# Autodesk Inventor assembly: Deltabot - Small Model ver12
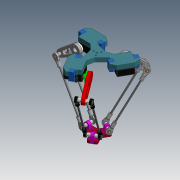
[picture p0: Inventor's stored thumbnail of the model, 180x180]
Saved by Autodesk Inventor 2014 SP1 (Build 180222100, 222)
## iProperties
Created: 2013-12-25
Part Number: Deltabot - Small Model ver12
Document SubType Name: Assembly
Designer: tom
Title: D:\My Documents\Work\GitHub\Delta_Robots\Delatabot - Small Model\Deltabot - Small Model.stp
Creation Date: 2013-12-24
Sending System: ACIS
Author: tom
## Documents named in this file (7)
- C:\Users\tom\Documents\GitHub\Delta_Robots\Delatabot - Small Model\Inventor\Deltabot - Small Model ver12\Deltabot - Small Model ver12.iam
- C:\Users\tom\Documents\GitHub\Vacubot\Inventor\Part2.ipt
- C:\Users\tom\Documents\GitHub\Delta_Robots\Delatabot - Small Model\Inventor\Deltabot - Small Model ver12\Servo_Mount.ipt
- C:\Users\tom\Documents\GitHub\Delta_Robots\Delatabot - Small Model\Inventor\Deltabot - Small Model ver12\Servo.ipt
- C:\Users\tom\Documents\GitHub\Delta_Robots\Delatabot - Small Model\Inventor\Deltabot - Small Model ver12\Servo Arm.iam
- C:\Users\tom\Documents\GitHub\Delta_Robots\Delatabot - Small Model\Inventor\Deltabot - Small Model ver12\Arm Linkage.iam
- C:\Users\tom\Documents\GitHub\Delta_Robots\Delatabot - Small Model\Inventor\Deltabot - Small Model ver12\Lower Platform Assembly.iam
## Components (20 placed, 6 different names)
1. Upper Support — Mate:15, Mate:16, Mate:17, Mate:19
2. Servo Arm:1 [sub-assembly] — Ball:1, Ball:3
3. Arm Linkage:1 [sub-assembly] — Ball:1, Ball:2
4. Lower Platform Assembly:1 [sub-assembly] — Ball:2, Ball:4, Ball:6, Ball:8, Ball:10, Ball:12
5. Arm Linkage:2 [sub-assembly] — Ball:3, Ball:4
6. Servo Arm:2 [sub-assembly] — Rotational:2, Ball:5, Ball:7
7. Arm Linkage:3 [sub-assembly] — Ball:5, Ball:6
8. Arm Linkage:4 [sub-assembly] — Ball:7, Ball:8
9. Servo Arm:3 [sub-assembly] — Rotational:3, Ball:9, Ball:11
10. Arm Linkage:5 [sub-assembly] — Ball:9, Ball:10
11. Arm Linkage:6 [sub-assembly] — Ball:11, Ball:12
12. Servo_Mount:1 — Mate:16, Mate:17, Mate:18, Mate:20
13. Servo_Mount:2 — Mate:15, Mate:19, Mate:21
14. Servo:1 — Mate:18, Mate:20, Mate:21
15. Servo_Mount:3
16. Servo_Mount:4
17. Servo:2 — Rotational:3
18. Servo_Mount:5
19. Servo_Mount:6
20. Servo:3 — Rotational:2
## Component patterns: (3 elements, first: Servo_Mount:1 + Servo_Mount:2 + Servo:1)
## Relationships (22: BallJoint 12, Mate 7, RevoluteJoint 3)
- Mate:15: Upper Support ↔ Servo_Mount:2
- Mate:16: Upper Support ↔ Servo_Mount:1
- Mate:17: Upper Support ↔ Servo_Mount:1
- Mate:18: Servo_Mount:1 ↔ Servo:1
- Mate:19: Upper Support ↔ Servo_Mount:2
- Mate:20: Servo_Mount:1 ↔ Servo:1
- Mate:21 (0.005 mm): Servo_Mount:2 ↔ Servo:1
- [RevoluteJoint]: Servo Arm:1 ↔ Servo:1
- Ball:1: Servo Arm:1 ↔ Arm Linkage:1
- Ball:2: Arm Linkage:1 ↔ Lower Platform Assembly:1
- Ball:3: Servo Arm:1 ↔ Arm Linkage:2
- Ball:4: Lower Platform Assembly:1 ↔ Arm Linkage:2
- Rotational:2 [RevoluteJoint]: Servo Arm:2 ↔ Servo:3
- Ball:5: Servo Arm:2 ↔ Arm Linkage:3
- Ball:6: Lower Platform Assembly:1 ↔ Arm Linkage:3
- Ball:7: Servo Arm:2 ↔ Arm Linkage:4
- Ball:8: Lower Platform Assembly:1 ↔ Arm Linkage:4
- Rotational:3 [RevoluteJoint]: Servo Arm:3 ↔ Servo:2
- Ball:9: Servo Arm:3 ↔ Arm Linkage:5
- Ball:10: Lower Platform Assembly:1 ↔ Arm Linkage:5
- Ball:11: Servo Arm:3 ↔ Arm Linkage:6
- Ball:12: Lower Platform Assembly:1 ↔ Arm Linkage:6
